# Autodesk Inventor assembly: Rocket_MK_II_assembly
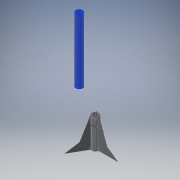
[picture p0: Inventor's stored thumbnail of the model, 180x180]
Saved by Autodesk Inventor 2017 (Build 210142000, 142)
## iProperties
Created: 2017-05-17
Part Number: Rocket_MK_II_assembly
Document SubType Name: Assembly
Designer: Harrison
Author: Harrison
## Documents named in this file (4)
- C:\Users\Harrison\Documents\AutoDesk\Rocket_MK_II_assembly.iam
- C:\Users\Harrison\Documents\AutoDesk\Engine_Holder_Mk_III_Good.ipt
- C:\Users\Harrison\Documents\AutoDesk\Rocket_MK_II_Fins_III.ipt
- C:\Users\Harrison\Documents\AutoDesk\Rocket_MK_II_housing.ipt
## Components (5 placed, 3 different names)
1. Engine_Holder_Mk_III_Good:1 — Mate:1, Flush:1, Rotational:1, Mate:2, Flush:2, Rotational:2, Mate:3, Flush:3, Rotational:3
2. Rocket_MK_II_Fins_III:1 — Mate:3, Flush:3, Rotational:3
3. Rocket_MK_II_Fins_III:2 — Mate:2, Flush:2, Rotational:2
4. Rocket_MK_II_Fins_III:3 — Mate:1, Flush:1, Rotational:1
5. Rocket_MK_II_housing:1
## Relationships (9: Mate 3, Flush 3, RevoluteJoint 3)
- Mate:1: Engine_Holder_Mk_III_Good:1 ↔ Rocket_MK_II_Fins_III:3
- Flush:1: Engine_Holder_Mk_III_Good:1 ↔ Rocket_MK_II_Fins_III:3
- Rotational:1 [RevoluteJoint]: Engine_Holder_Mk_III_Good:1 ↔ Rocket_MK_II_Fins_III:3
- Mate:2: Engine_Holder_Mk_III_Good:1 ↔ Rocket_MK_II_Fins_III:2
- Flush:2: Engine_Holder_Mk_III_Good:1 ↔ Rocket_MK_II_Fins_III:2
- Rotational:2 [RevoluteJoint]: Engine_Holder_Mk_III_Good:1 ↔ Rocket_MK_II_Fins_III:2
- Mate:3: Engine_Holder_Mk_III_Good:1 ↔ Rocket_MK_II_Fins_III:1
- Flush:3: Engine_Holder_Mk_III_Good:1 ↔ Rocket_MK_II_Fins_III:1
- Rotational:3 [RevoluteJoint]: Engine_Holder_Mk_III_Good:1 ↔ Rocket_MK_II_Fins_III:1
